# Autodesk Inventor assembly: Electromagnet final
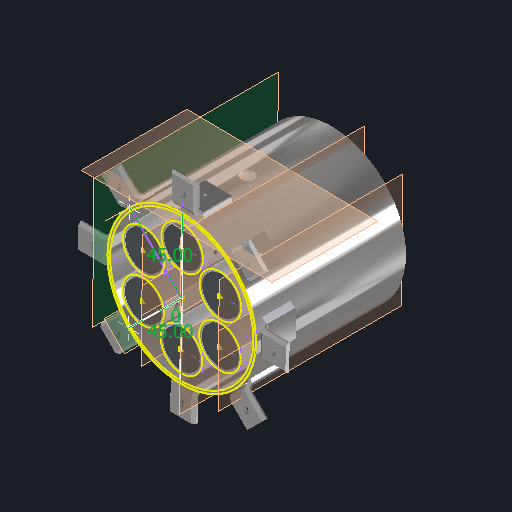
[picture p0: Inventor's stored thumbnail of the model, 512x512]
Saved by Autodesk Inventor 2026.3 (Build 303398000, 398)
## iProperties
Created: 2026-08-03
Part Number: Electromagnet final
Document SubType Name: Weldment
Designer: matot
Weld Material: Welded Aluminum-6061
Author: matot
## Documents named in this file (3)
- C:\Users\matot\OneDrive - Stellenbosch University\2026\MechatronicsProject478\Building the joint\Joint Assembly\Electromagnet final.iam
- C:\Users\matot\OneDrive - Stellenbosch University\2026\MechatronicsProject478\Building the joint\Joint Assembly\Electromagnet.iam
- C:\Users\matot\OneDrive - Stellenbosch University\2026\MechatronicsProject478\Building the joint\Joint Assembly\Pressure plate tab_L.ipt
## Components (9 placed, 2 different names)
1. Electromagnet:1 [sub-assembly] — Mate:1, Tangent:1, Mate:2, Tangent:2, Tangent:3, Mate:3, Flush:1, Tangent:4, Mate:4, Flush:2, Flush:3, Flush:4, Tangent:5, Mate:5, Flush:5, Tangent:6, Mate:6, Flush:6, Tangent:7, Mate:7, Flush:7, Tangent:8, Mate:8, Flush:8
2. Pressure plate tab_L:1 — Mate:2, Tangent:2, Flush:4
3. Pressure plate tab_L:2 — Mate:1, Tangent:1, Flush:3
4. Pressure plate tab_L:3 — Tangent:3, Mate:3, Flush:1
5. Pressure plate tab_L:4 — Tangent:4, Mate:4, Flush:2
6. Pressure plate tab_L:5 — Tangent:6, Mate:6, Flush:6
7. Pressure plate tab_L:6 — Tangent:7, Mate:7, Flush:7
8. Pressure plate tab_L:7 — Tangent:8, Mate:8, Flush:8
9. Pressure plate tab_L:8 — Tangent:5, Mate:5, Flush:5
## Relationships (24: Mate 8, Tangent 8, Flush 8)
- Mate:1: Electromagnet:1 ↔ Pressure plate tab_L:2
- Tangent:1: Electromagnet:1 ↔ Pressure plate tab_L:2
- Mate:2: Electromagnet:1 ↔ Pressure plate tab_L:1
- Tangent:2: Electromagnet:1 ↔ Pressure plate tab_L:1
- Tangent:3: Electromagnet:1 ↔ Pressure plate tab_L:3
- Mate:3: Electromagnet:1 ↔ Pressure plate tab_L:3
- Flush:1: Electromagnet:1 ↔ Pressure plate tab_L:3
- Tangent:4: Electromagnet:1 ↔ Pressure plate tab_L:4
- Mate:4: Electromagnet:1 ↔ Pressure plate tab_L:4
- Flush:2: Electromagnet:1 ↔ Pressure plate tab_L:4
- Flush:3: Electromagnet:1 ↔ Pressure plate tab_L:2
- Flush:4: Electromagnet:1 ↔ Pressure plate tab_L:1
- Tangent:5: Electromagnet:1 ↔ Pressure plate tab_L:8
- Mate:5: Electromagnet:1 ↔ Pressure plate tab_L:8
- Flush:5: Electromagnet:1 ↔ Pressure plate tab_L:8
- Tangent:6: Electromagnet:1 ↔ Pressure plate tab_L:5
- Mate:6: Electromagnet:1 ↔ Pressure plate tab_L:5
- Flush:6: Electromagnet:1 ↔ Pressure plate tab_L:5
- Tangent:7: Electromagnet:1 ↔ Pressure plate tab_L:6
- Mate:7: Electromagnet:1 ↔ Pressure plate tab_L:6
- Flush:7: Electromagnet:1 ↔ Pressure plate tab_L:6
- Tangent:8: Electromagnet:1 ↔ Pressure plate tab_L:7
- Mate:8: Electromagnet:1 ↔ Pressure plate tab_L:7
- Flush:8: Electromagnet:1 ↔ Pressure plate tab_L:7
